# Autodesk Inventor assembly: BHSS
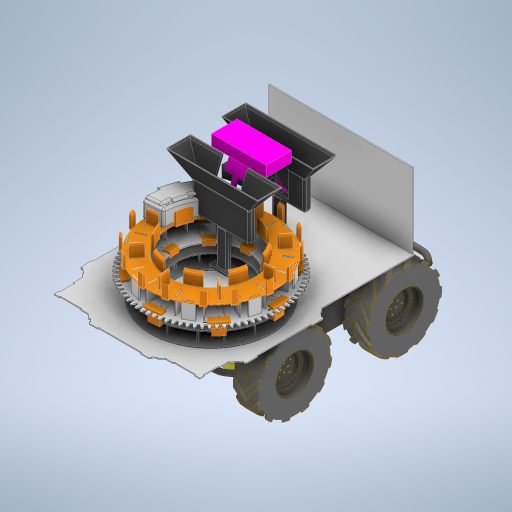
[picture p0: Inventor's stored thumbnail of the model, 512x512]
Saved by Autodesk Inventor 2023 (Build 270158000, 158)
## iProperties
Created: 2022-10-26
Part Number: BHSS
Document SubType Name: Assembly
Designer: cheng
Mass: 107138 g
Surface Area: 105016 cm^2
Volume: 89092.4 cm^3
Density: 1.20255 g/cm^3
Author: cheng
## Documents named in this file (10)
- C:\Users\mihal\Desktop\12a th Assembly\BHSS.iam
- C:\Users\mihal\Desktop\12a th Assembly\drone model.ipt
- C:\Users\mihal\Desktop\12a th Assembly\Husky_3D_Model.ipt
- C:\Users\mihal\Desktop\12a th Assembly\Inner Circle Landing Legs.ipt
- C:\Users\mihal\Desktop\12a th Assembly\Battery_Module_Second_Iteration.ipt
- Battery Module Second Iteration.ipt
- C:\Users\mihal\Desktop\12a th Assembly\Moving Carousel\Moving Carousel Assembly.iam
- C:\Users\mihal\Desktop\12a th Assembly\Carousel Base Plate Laser Cut\base Plate Laser Full Carou ASSEMBLY.iam
- C:\Users\mihal\Desktop\12a th Assembly\Base Plate V2\Base Plate Assembly.iam
- C:\Users\mihal\Desktop\12a th Assembly\Battery Cage and Spring Plate.iam
## Components (9 placed, 8 different names)
1. drone model:1 — Mate:124, Mate:125, Mate:126
2. Husky_3D_Model:1 — Flush:1
3. Inner Circle Landing Legs:2
4. Inner Circle Landing Legs:4
5. Battery Module Second Iteration:1 — Mate:121, Mate:122, Mate:123
6. Moving Carousel Assembly:1 [sub-assembly] — Mate:117, Mate:118, Mate:121, Mate:122, Mate:123, Angle:1
7. base Plate Laser Full Carou ASSEMBLY:1 [sub-assembly] — Mate:117, Mate:118, Mate:119, Angle:1
8. Base Plate Assembly:1 [sub-assembly] — Flush:1, Mate:119
9. Battery Cage and Spring Plate:1 [sub-assembly] — Mate:124, Mate:125, Mate:126
## Relationships (11: Mate 9, Flush 1, Angle 1)
- Mate:117: Moving Carousel Assembly:1 ↔ base Plate Laser Full Carou ASSEMBLY:1
- Mate:118: Moving Carousel Assembly:1 ↔ base Plate Laser Full Carou ASSEMBLY:1
- Flush:1: Husky_3D_Model:1 ↔ Base Plate Assembly:1
- Mate:119: base Plate Laser Full Carou ASSEMBLY:1 ↔ Base Plate Assembly:1
- Mate:121: Battery Module Second Iteration:1 ↔ Moving Carousel Assembly:1
- Mate:122 (20 mm): Battery Module Second Iteration:1 ↔ Moving Carousel Assembly:1
- Mate:123: Battery Module Second Iteration:1 ↔ Moving Carousel Assembly:1
- Mate:124: drone model:1 ↔ Battery Cage and Spring Plate:1
- Mate:125: drone model:1 ↔ Battery Cage and Spring Plate:1
- Mate:126: drone model:1 ↔ Battery Cage and Spring Plate:1
- Angle:1 (10 deg): Moving Carousel Assembly:1 ↔ base Plate Laser Full Carou ASSEMBLY:1
